# Autodesk Inventor assembly: Rail_Assembly
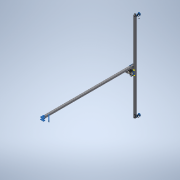
[picture p0: Inventor's stored thumbnail of the model, 180x180]
Saved by Autodesk Inventor 2021 (Build 250183000, 183)
## iProperties
Created: 2021-01-25
Part Number: Rail_Assembly
Document SubType Name: Assembly
Designer: Jorian Brusind
Mass: 3786.54 g
Surface Area: 19508.5 cm^2
Volume: 2323.9 cm^3
Density: 1.62939 g/cm^3
Author: Jorian Brusind
## Documents named in this file (26)
- C:\Users\Jorian Brusind\Documents\GitHub\PersonalProjects\HyperRail\Inventor Files\Rail_Assembly.iam
- C:\Users\Jorian Brusind\Documents\GitHub\PersonalProjects\Inventor Projects\Useful models\NEMA_Steppers\NEMA23\23HS8430B.ipt
- C:\Users\Jorian Brusind\Documents\GitHub\PersonalProjects\HyperRail\Inventor Files\NEMA23_StepperonlineMount.ipt
- C:\Users\Jorian Brusind\Documents\GitHub\PersonalProjects\HyperRail\Inventor Files\Roller_Bracket.iam
- C:\Users\Jorian Brusind\Documents\GitHub\PersonalProjects\Inventor Projects\Useful models\8020_Sets\IPT_20_Series\IPT_20_Series\20-2040_200mm.ipt
- C:\Users\Jorian Brusind\Documents\GitHub\PersonalProjects\HyperRail\Inventor Files\2804S_NEMA2115_1Gearbox.ipt
- C:\Users\Jorian Brusind\Documents\GitHub\PersonalProjects\Inventor Projects\Useful models\8020_Sets\IPT_40_Series\Extra_40_Series\90deg_4040.ipt
- C:\Users\Jorian Brusind\Documents\GitHub\PersonalProjects\HyperRail\Inventor Files\SmallBelt_LargePulley.ipt
- C:\Users\Jorian Brusind\Documents\GitHub\PersonalProjects\HyperRail\Inventor Files\11mm_BearingWheel.ipt
- C:\Users\Jorian Brusind\Documents\GitHub\PersonalProjects\Inventor Projects\Useful models\Metric bolt\Bolt M5 25mm.ipt
- C:\Users\Jorian Brusind\Documents\GitHub\PersonalProjects\HyperRail\Inventor Files\Small_belt_5mm_1mm.ipt
- C:\Users\Jorian Brusind\Documents\GitHub\PersonalProjects\Inventor Projects\Useful models\8020_Sets\IPT_20_Series\Extra_20_Series\8020_14056m\14056_m.ipt
- C:\Users\Jorian Brusind\Documents\GitHub\PersonalProjects\HyperRail\PCB Files\Integrated Stepper Motor Driver\ExportSTEP\Main.iam
- C:\Users\Jorian Brusind\Documents\GitHub\PersonalProjects\HyperRail\Inventor Files\NEMA23_Shroud.ipt
- C:\Users\Jorian Brusind\Documents\GitHub\PersonalProjects\Inventor Projects\Useful models\8020_Sets\IPT_20_Series\IPT_20_Series\20-4040_2m.ipt
- C:\Users\Jorian Brusind\Documents\GitHub\PersonalProjects\HyperRail\Inventor Files\98952A059_ALUM MALE-FEM THRDED HEX STANDOFF.ipt
- C:\Users\Jorian Brusind\Documents\GitHub\PersonalProjects\HyperRail\Inventor Files\95783A039_NYLON 6-6 MALE-FEM THRDED HEX STANDOFF.ipt
- C:\Users\Jorian Brusind\Documents\GitHub\PersonalProjects\HyperRail\Inventor Files\Integrated_Stepper_NEMA23_Mount.ipt
- C:\Users\Jorian Brusind\Documents\GitHub\PersonalProjects\HyperRail\Inventor Files\4mm_Roller_Spacer.ipt
- C:\Users\Jorian Brusind\Documents\GitHub\PersonalProjects\HyperRail\Inventor Files\Foot_Spacer.ipt
- C:\Users\Jorian Brusind\Documents\GitHub\PersonalProjects\Inventor Projects\Useful models\Metric bolt\Bolt M5 50mm.ipt
- C:\Users\Jorian Brusind\Documents\GitHub\PersonalProjects\Inventor Projects\Useful models\Metric nuts\Nut M5.ipt
- C:\Users\Jorian Brusind\Documents\GitHub\PersonalProjects\HyperRail\Inventor Files\Bottom_Foot.ipt
- C:\Users\Jorian Brusind\Documents\GitHub\PersonalProjects\HyperRail\Inventor Files\120deg_Tslot_Gusset.ipt
- C:\Users\Jorian Brusind\Documents\GitHub\PersonalProjects\HyperRail\Inventor Files\90deg_4040Bracket.ipt
- C:\Users\Jorian Brusind\Documents\GitHub\PersonalProjects\HyperRail\Inventor Files\Belt_Washer.ipt
## Components (48 placed, 25 different names)
1. 23HS8430B:1 — Mate:127, Angle:3, Mate:158, Mate:175, Mate:176, Mate:177, Mate:179, Mate:180, Mate:181, Mate:182, Mate:183, Mate:184, Mate:185, Mate:196
2. NEMA23_StepperonlineMount:1 — Angle:2, Mate:98, Mate:101, Mate:128, Mate:149, Mate:155, Flush:65, Mate:209, Mate:212, Mate:214
3. Roller_Bracket:1 [sub-assembly] — Flush:45, Mate:113, Mate:117, Flush:50, Mate:120, Flush:51, Mate:141, Flush:57
4. Roller_Bracket:2 [sub-assembly] — Flush:57, Mate:142, Flush:58, Mate:143, Mate:144, Mate:145
5. 20-2040_200mm:1 — Flush:34, Mate:83, Flush:35, Flush:36, Mate:85, Flush:45, Mate:113, Mate:118, Mate:119, Mate:121, Mate:124, Flush:56, Mate:142, Flush:58, Flush:59, Flush:60, Flush:63, Mate:151
6. 2804S_NEMA2115_1Gearbox:1 — Angle:2, Mate:98, Mate:109, Mate:127, Mate:128, Angle:3, Mate:158, Mate:204, Flush:66
7. 90deg_4040:1 — Flush:34, Mate:83, Flush:35, Mate:150
8. 90deg_4040:2 — Flush:36, Mate:85, Mate:149, Mate:152
9. SmallBelt_LargePulley:1 — Mate:204, Flush:66
10. 11mm_BearingWheel:1 — Mate:101, Mate:102, Mate:242
11. Bolt M5 25mm:1 — Mate:102, Mate:213, Mate:241
12. Small_belt_5mm_1mm:1 — Mate:109, Flush:42, Mate:111, Flush:64
13. Small_belt_5mm_1mm:2 — Flush:42, Mate:111, Mate:154, Flush:64, Mate:205
14. 14056_m:1 — Mate:117, Mate:118, Flush:50
15. 14056_m:2 — Mate:119, Mate:120, Flush:51
16. 14056_m:3 — Mate:121, Mate:144, Flush:60
17. 14056_m:4 — Mate:124, Mate:143, Flush:59
18. Main:1 [sub-assembly] — Mate:199, Mate:202, Mate:203
19. 20-4040_2m:1 — Mate:139, Mate:140, Mate:141, Flush:56, Mate:145, Mate:154, Mate:205, Mate:243, Flush:76, Flush:77, Mate:248, Flush:79, Flush:80
20. 20-4040_2m:2 — Mate:150, Flush:63, Mate:151, Mate:152, Mate:155, Flush:65, Mate:230, Flush:69, Flush:70, Mate:231, Flush:71, Flush:72, Mate:232, Flush:73, Mate:233, Mate:234, Flush:74
21. NEMA23_Shroud:1 — Mate:175, Mate:176, Mate:201
22. 98952A059_ALUM MALE-FEM THRDED HEX STANDOFF:1 — Mate:180, Mate:181, Mate:186, Mate:191
23. 98952A059_ALUM MALE-FEM THRDED HEX STANDOFF:2 — Mate:184, Mate:185, Mate:189, Mate:192
24. 98952A059_ALUM MALE-FEM THRDED HEX STANDOFF:3 — Mate:177, Mate:179, Mate:187, Mate:190
25. 98952A059_ALUM MALE-FEM THRDED HEX STANDOFF:4 — Mate:182, Mate:183, Mate:188, Mate:193
26. 95783A039_NYLON 6-6 MALE-FEM THRDED HEX STANDOFF:1 — Mate:188, Mate:193, Angle:4
27. 95783A039_NYLON 6-6 MALE-FEM THRDED HEX STANDOFF:2 — Mate:186, Mate:191
28. 95783A039_NYLON 6-6 MALE-FEM THRDED HEX STANDOFF:3 — Mate:187, Mate:190, Mate:200
29. 95783A039_NYLON 6-6 MALE-FEM THRDED HEX STANDOFF:4 — Mate:189, Mate:192
30. Integrated_Stepper_NEMA23_Mount:1 — Mate:196, Mate:199, Mate:200, Mate:201, Mate:202, Mate:203, Angle:4
31. 11mm_BearingWheel:2 — Mate:237, Mate:240
32. Bolt M5 25mm:2 — Mate:209, Mate:210, Mate:235, Mate:238, Mate:239
33. 4mm_Roller_Spacer:1 — Mate:210, Mate:212, Mate:236
34. 4mm_Roller_Spacer:2 — Mate:213, Mate:214, Mate:252
35. Bolt M5 50mm:1 — Mate:224, Mate:245, Mate:246, Mate:247
36. Nut M5:1 — Mate:226, Mate:247
37. Nut M5:2 — Mate:244, Flush:78, Mate:246
38. Bottom_Foot:1 — Mate:224, Mate:226, Mate:245, Flush:81
39. 120deg_Tslot_Gusset:1 — Mate:230, Flush:69, Flush:70
40. 120deg_Tslot_Gusset:2 — Mate:231, Flush:71, Flush:72
41. 90deg_4040Bracket:1 — Mate:232, Flush:73, Mate:233, Flush:75
42. 90deg_4040Bracket:2 — Mate:234, Flush:74, Flush:75
43. Belt_Washer:1 — Mate:238, Mate:239, Mate:240, Mate:241
44. Belt_Washer:2 — Mate:235, Mate:236, Mate:237, Mate:242, Mate:252
45. Foot_Spacer:1 — Mate:243, Flush:76, Flush:77, Mate:244, Flush:78
46. Foot_Spacer:2 — Mate:248, Flush:79, Flush:80, Mate:250
47. Bottom_Foot:2 — Mate:249, Mate:251, Flush:81
48. Bolt M5 50mm:2 — Mate:249, Mate:250, Mate:251
## Relationships (119: Mate 87, Flush 29, Angle 3)
- Angle:2 (0 deg): NEMA23_StepperonlineMount:1 ↔ 2804S_NEMA2115_1Gearbox:1
- Flush:34: 20-2040_200mm:1 ↔ 90deg_4040:1
- Mate:83: 20-2040_200mm:1 ↔ 90deg_4040:1
- Flush:35: 20-2040_200mm:1 ↔ 90deg_4040:1
- Flush:36: 20-2040_200mm:1 ↔ 90deg_4040:2
- Mate:85: 20-2040_200mm:1 ↔ 90deg_4040:2
- Mate:98: NEMA23_StepperonlineMount:1 ↔ 2804S_NEMA2115_1Gearbox:1
- Mate:101: NEMA23_StepperonlineMount:1 ↔ 11mm_BearingWheel:1
- Mate:102: 11mm_BearingWheel:1 ↔ Bolt M5 25mm:1
- Mate:109 (10 mm): 2804S_NEMA2115_1Gearbox:1 ↔ Small_belt_5mm_1mm:1
- Flush:42: Small_belt_5mm_1mm:1 ↔ Small_belt_5mm_1mm:2
- Mate:111 (20 mm): Small_belt_5mm_1mm:1 ↔ Small_belt_5mm_1mm:2
- Flush:45: Roller_Bracket:1 ↔ 20-2040_200mm:1
- Mate:113: Roller_Bracket:1 ↔ 20-2040_200mm:1
- Mate:117: Roller_Bracket:1 ↔ 14056_m:1
- Mate:118: 20-2040_200mm:1 ↔ 14056_m:1
- Flush:50: Roller_Bracket:1 ↔ 14056_m:1
- Mate:119: 20-2040_200mm:1 ↔ 14056_m:2
- Mate:120: Roller_Bracket:1 ↔ 14056_m:2
- Flush:51: Roller_Bracket:1 ↔ 14056_m:2
- Mate:121: 20-2040_200mm:1 ↔ 14056_m:3
- Mate:124: 20-2040_200mm:1 ↔ 14056_m:4
- Mate:127: 23HS8430B:1 ↔ 2804S_NEMA2115_1Gearbox:1
- Mate:128: NEMA23_StepperonlineMount:1 ↔ 2804S_NEMA2115_1Gearbox:1
- Mate:139: 20-4040_2m:1
- Mate:140: 20-4040_2m:1
- Mate:141 (11 mm): Roller_Bracket:1 ↔ 20-4040_2m:1
- Flush:56: 20-2040_200mm:1 ↔ 20-4040_2m:1
- Flush:57: Roller_Bracket:1 ↔ Roller_Bracket:2
- Mate:142: Roller_Bracket:2 ↔ 20-2040_200mm:1
- Flush:58: Roller_Bracket:2 ↔ 20-2040_200mm:1
- Mate:143: Roller_Bracket:2 ↔ 14056_m:4
- Flush:59: 20-2040_200mm:1 ↔ 14056_m:4
- Mate:144: Roller_Bracket:2 ↔ 14056_m:3
- Flush:60: 20-2040_200mm:1 ↔ 14056_m:3
- Mate:145 (8 mm): Roller_Bracket:2 ↔ 20-4040_2m:1
- Mate:149 (5 mm): NEMA23_StepperonlineMount:1 ↔ 90deg_4040:2
- Mate:150: 90deg_4040:1 ↔ 20-4040_2m:2
- Flush:63: 20-2040_200mm:1 ↔ 20-4040_2m:2
- Mate:151: 20-2040_200mm:1 ↔ 20-4040_2m:2
- Mate:152: 90deg_4040:2 ↔ 20-4040_2m:2
- Mate:154 (-10 mm): Small_belt_5mm_1mm:2 ↔ 20-4040_2m:1
- Flush:64: Small_belt_5mm_1mm:1 ↔ Small_belt_5mm_1mm:2
- Mate:155: NEMA23_StepperonlineMount:1 ↔ 20-4040_2m:2
- Flush:65 (18 mm): NEMA23_StepperonlineMount:1 ↔ 20-4040_2m:2
- Angle:3 (0 deg): 23HS8430B:1 ↔ 2804S_NEMA2115_1Gearbox:1
- Mate:158: 23HS8430B:1 ↔ 2804S_NEMA2115_1Gearbox:1
- Mate:175 (1 mm): 23HS8430B:1 ↔ NEMA23_Shroud:1
- Mate:176 (1 mm): 23HS8430B:1 ↔ NEMA23_Shroud:1
- Mate:177: 23HS8430B:1 ↔ 98952A059_ALUM MALE-FEM THRDED HEX STANDOFF:3
- Mate:179: 23HS8430B:1 ↔ 98952A059_ALUM MALE-FEM THRDED HEX STANDOFF:3
- Mate:180: 23HS8430B:1 ↔ 98952A059_ALUM MALE-FEM THRDED HEX STANDOFF:1
- Mate:181: 23HS8430B:1 ↔ 98952A059_ALUM MALE-FEM THRDED HEX STANDOFF:1
- Mate:182: 23HS8430B:1 ↔ 98952A059_ALUM MALE-FEM THRDED HEX STANDOFF:4
- Mate:183: 23HS8430B:1 ↔ 98952A059_ALUM MALE-FEM THRDED HEX STANDOFF:4
- Mate:184: 23HS8430B:1 ↔ 98952A059_ALUM MALE-FEM THRDED HEX STANDOFF:2
- Mate:185: 23HS8430B:1 ↔ 98952A059_ALUM MALE-FEM THRDED HEX STANDOFF:2
- Mate:186: 98952A059_ALUM MALE-FEM THRDED HEX STANDOFF:1 ↔ 95783A039_NYLON 6-6 MALE-FEM THRDED HEX STANDOFF:2
- Mate:187: 98952A059_ALUM MALE-FEM THRDED HEX STANDOFF:3 ↔ 95783A039_NYLON 6-6 MALE-FEM THRDED HEX STANDOFF:3
- Mate:188: 98952A059_ALUM MALE-FEM THRDED HEX STANDOFF:4 ↔ 95783A039_NYLON 6-6 MALE-FEM THRDED HEX STANDOFF:1
- Mate:189: 98952A059_ALUM MALE-FEM THRDED HEX STANDOFF:2 ↔ 95783A039_NYLON 6-6 MALE-FEM THRDED HEX STANDOFF:4
- Mate:190: 98952A059_ALUM MALE-FEM THRDED HEX STANDOFF:3 ↔ 95783A039_NYLON 6-6 MALE-FEM THRDED HEX STANDOFF:3
- Mate:191: 98952A059_ALUM MALE-FEM THRDED HEX STANDOFF:1 ↔ 95783A039_NYLON 6-6 MALE-FEM THRDED HEX STANDOFF:2
- Mate:192: 98952A059_ALUM MALE-FEM THRDED HEX STANDOFF:2 ↔ 95783A039_NYLON 6-6 MALE-FEM THRDED HEX STANDOFF:4
- Mate:193: 98952A059_ALUM MALE-FEM THRDED HEX STANDOFF:4 ↔ 95783A039_NYLON 6-6 MALE-FEM THRDED HEX STANDOFF:1
- Mate:196 (2 mm): 23HS8430B:1 ↔ Integrated_Stepper_NEMA23_Mount:1
- Mate:199 (1 mm): Main:1 ↔ Integrated_Stepper_NEMA23_Mount:1
- Mate:200: 95783A039_NYLON 6-6 MALE-FEM THRDED HEX STANDOFF:3 ↔ Integrated_Stepper_NEMA23_Mount:1
- Mate:201: NEMA23_Shroud:1 ↔ Integrated_Stepper_NEMA23_Mount:1
- Mate:202: Main:1 ↔ Integrated_Stepper_NEMA23_Mount:1
- Mate:203: Main:1 ↔ Integrated_Stepper_NEMA23_Mount:1
- Angle:4 (0 deg): 95783A039_NYLON 6-6 MALE-FEM THRDED HEX STANDOFF:1 ↔ Integrated_Stepper_NEMA23_Mount:1
- Mate:204: 2804S_NEMA2115_1Gearbox:1 ↔ SmallBelt_LargePulley:1
- Flush:66 (3 mm): 2804S_NEMA2115_1Gearbox:1 ↔ SmallBelt_LargePulley:1
- Mate:205: Small_belt_5mm_1mm:2 ↔ 20-4040_2m:1
- [Mate]: 11mm_BearingWheel:2 ↔ Bolt M5 25mm:2
- Mate:209: NEMA23_StepperonlineMount:1 ↔ Bolt M5 25mm:2
- Mate:210: Bolt M5 25mm:2 ↔ 4mm_Roller_Spacer:1
- Mate:212: NEMA23_StepperonlineMount:1 ↔ 4mm_Roller_Spacer:1
- Mate:213: Bolt M5 25mm:1 ↔ 4mm_Roller_Spacer:2
- Mate:214: NEMA23_StepperonlineMount:1 ↔ 4mm_Roller_Spacer:2
- Mate:224: Bolt M5 50mm:1 ↔ Bottom_Foot:1
- Mate:226: Nut M5:1 ↔ Bottom_Foot:1
- Mate:230: 20-4040_2m:2 ↔ 120deg_Tslot_Gusset:1
- Flush:69: 20-4040_2m:2 ↔ 120deg_Tslot_Gusset:1
- Flush:70: 20-4040_2m:2 ↔ 120deg_Tslot_Gusset:1
- Mate:231: 20-4040_2m:2 ↔ 120deg_Tslot_Gusset:2
- Flush:71: 20-4040_2m:2 ↔ 120deg_Tslot_Gusset:2
- Flush:72: 20-4040_2m:2 ↔ 120deg_Tslot_Gusset:2
- Mate:232: 20-4040_2m:2 ↔ 90deg_4040Bracket:1
- Flush:73: 20-4040_2m:2 ↔ 90deg_4040Bracket:1
- Mate:233: 20-4040_2m:2 ↔ 90deg_4040Bracket:1
- Mate:234: 20-4040_2m:2 ↔ 90deg_4040Bracket:2
- Flush:74: 20-4040_2m:2 ↔ 90deg_4040Bracket:2
- Flush:75: 90deg_4040Bracket:1 ↔ 90deg_4040Bracket:2
- Mate:235: Bolt M5 25mm:2 ↔ Belt_Washer:2
- Mate:236: 4mm_Roller_Spacer:1 ↔ Belt_Washer:2
- Mate:237: 11mm_BearingWheel:2 ↔ Belt_Washer:2
- Mate:238: Bolt M5 25mm:2 ↔ Belt_Washer:1
- Mate:239: Bolt M5 25mm:2 ↔ Belt_Washer:1
- Mate:240: 11mm_BearingWheel:2 ↔ Belt_Washer:1
- Mate:241: Bolt M5 25mm:1 ↔ Belt_Washer:1
- Mate:242: 11mm_BearingWheel:1 ↔ Belt_Washer:2
- Mate:243: 20-4040_2m:1 ↔ Foot_Spacer:1
- Flush:76: 20-4040_2m:1 ↔ Foot_Spacer:1
- Flush:77: 20-4040_2m:1 ↔ Foot_Spacer:1
- Mate:244: Nut M5:2 ↔ Foot_Spacer:1
- Flush:78: Nut M5:2 ↔ Foot_Spacer:1
- Mate:245: Bolt M5 50mm:1 ↔ Bottom_Foot:1
- Mate:246: Bolt M5 50mm:1 ↔ Nut M5:2
- Mate:247: Bolt M5 50mm:1 ↔ Nut M5:1
- Mate:248: 20-4040_2m:1 ↔ Foot_Spacer:2
- Flush:79: 20-4040_2m:1 ↔ Foot_Spacer:2
- Flush:80: 20-4040_2m:1 ↔ Foot_Spacer:2
- Mate:249: Bottom_Foot:2 ↔ Bolt M5 50mm:2
- Mate:250: Foot_Spacer:2 ↔ Bolt M5 50mm:2
- Mate:251: Bottom_Foot:2 ↔ Bolt M5 50mm:2
- Flush:81: Bottom_Foot:1 ↔ Bottom_Foot:2
- Mate:252: 4mm_Roller_Spacer:2 ↔ Belt_Washer:2
## Named parameters: d352_d202 = 0 mm
